# Autodesk Inventor assembly: Euph Mellie Combo Cart
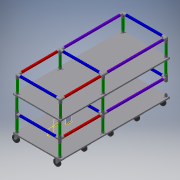
[picture p0: Inventor's stored thumbnail of the model, 180x180]
Saved by Autodesk Inventor 2018.2 (Build 222227000, 227)
## iProperties
Created: 2018-02-07
Part Number: Euph Mellie Combo Cart
Document SubType Name: Assembly
Designer: owner
Author: owner
## Documents named in this file (13)
- Z:\The Pickle\Final Carts\Euph Cart\Euph Mellie Combo Cart.iam
- Z:\The Pickle\Final Carts\Euph Cart\Plywood Base.ipt
- Z:\The Pickle\Inventor Pipe Parts\Formufit Fittings\4-way Tee 1 Inch.ipt
- Z:\The Pickle\Inventor Pipe Parts\Formufit Fittings\Tee 1 Inch.ipt
- Z:\The Pickle\Inventor Pipe Parts\Formufit Fittings\Wood Mount 1 Inch.ipt
- Z:\The Pickle\Final Carts\Euph Cart\Pipe 1.ipt
- Z:\The Pickle\Final Carts\Euph Cart\Pipe 2.ipt
- Z:\The Pickle\Final Carts\Euph Cart\Pipe 3.ipt
- Z:\The Pickle\Final Carts\Euph Cart\Pipe 4.ipt
- Z:\The Pickle\Inventor Pipe Parts\Formufit Fittings\5-way 1 Inch.ipt
- Z:\The Pickle\Inventor Pipe Parts\Formufit Fittings\3-way 90 1 Inch.ipt
- Z:\The Pickle\Final Carts\Eye Bolt and Nut.iam
- Z:\The Pickle\Final Carts\WHEELS.ipt
## Components (76 placed, 12 different names)
1. Plywood Base:1 — Mate:2, Tangent:1, Tangent:2, Tangent:3, Flush:1, Flush:2, Mate:6, Tangent:7, Tangent:8, Tangent:9, Tangent:10, Tangent:11, Mate:14, Flush:36, Flush:37, Flush:38
2. Plywood Base:2 — Mate:3, Mate:4, Tangent:4, Tangent:5, Tangent:6, Flush:1, Flush:2
3. Pipe 1:1 — Insert:47
4. Pipe 1:2 — Insert:48
5. Pipe 1:3 — Insert:41, Insert:42
6. Pipe 1:4 — Insert:9, Insert:10
7. Pipe 1:5 — Insert:11, Insert:12
8. Pipe 1:6 — Insert:3, Insert:4
9. Pipe 2:1 — Insert:45, Insert:46
10. Pipe 2:2 — Insert:37, Insert:38
11. Pipe 2:3 — Insert:5, Insert:6
12. Pipe 3:1 — Insert:13, Insert:30
13. Pipe 3:2 — Insert:14, Insert:33
14. Pipe 3:3 — Insert:1, Insert:2
15. Pipe 3:4 — Insert:15, Insert:34
16. Pipe 3:5 — Insert:17, Insert:31
17. Pipe 3:6 — Insert:18, Insert:26
18. Pipe 3:7 — Insert:16, Insert:32
19. Pipe 3:8 — Insert:19, Insert:29
20. Pipe 3:9 — Insert:21, Insert:27
21. Pipe 3:10 — Insert:20, Insert:25
22. Pipe 3:11 — Insert:22, Insert:28
23. Pipe 3:12 — Insert:23, Insert:24
24. Pipe 4:1 — Insert:39, Insert:40
25. Pipe 4:2 — Insert:7, Insert:8
26. Pipe 4:3 — Insert:43, Insert:44
27. Wood Mount 1 Inch:1 — Insert:54
28. Wood Mount 1 Inch:2 — Insert:34, Tangent:10, Tangent:11
29. Wood Mount 1 Inch:3 — Mate:4, Tangent:4, Tangent:5, Tangent:6, Insert:35
30. Wood Mount 1 Inch:4 — Insert:33
31. Wood Mount 1 Inch:5 — Insert:56
32. Wood Mount 1 Inch:6 — Insert:58
33. Wood Mount 1 Inch:7 — Insert:24, Mate:3
34. Wood Mount 1 Inch:8 — Insert:25
35. Wood Mount 1 Inch:9 — Insert:26
36. Wood Mount 1 Inch:10 — Insert:29
37. Wood Mount 1 Inch:11 — Insert:27
38. Wood Mount 1 Inch:12 — Insert:28, Mate:6, Tangent:7, Tangent:8, Tangent:9
39. Wood Mount 1 Inch:13 — Insert:30
40. Wood Mount 1 Inch:14 — Mate:2, Tangent:1, Tangent:2, Tangent:3, Insert:1
41. Wood Mount 1 Inch:15 — Insert:32
42. Wood Mount 1 Inch:16 — Insert:31
43. Wood Mount 1 Inch:17 — Insert:55
44. Wood Mount 1 Inch:18 — Insert:57
45. 3-way 90 1 Inch:1 — Insert:40, Insert:41, Insert:50
46. 3-way 90 1 Inch:2 — Insert:36, Insert:37
47. 3-way 90 1 Inch:3 — Insert:46, Insert:47, Insert:53
48. 3-way 90 1 Inch:4 — Insert:42, Insert:43, Insert:51
49. 4-way Tee 1 Inch:1 — Insert:38, Insert:39, Insert:49
50. 4-way Tee 1 Inch:2 — Insert:44, Insert:45, Insert:48, Insert:52
51. 4-way Tee 1 Inch:3 — Insert:4, Insert:5, Insert:13, Insert:20
52. 4-way Tee 1 Inch:4 — Insert:8, Insert:9, Insert:15, Insert:21
53. 5-way 1 Inch:2 — Insert:6, Insert:7, Insert:11, Insert:14, Insert:18
54. Tee 1 Inch:1 — Insert:10, Insert:16, Insert:22
55. Tee 1 Inch:2 — Insert:2, Insert:3, Insert:23
56. Tee 1 Inch:3 — Insert:12, Insert:17, Insert:19
57. Pipe 3:13 — Insert:53, Insert:54
58. Pipe 3:14 — Insert:50, Insert:58
59. Pipe 3:15 — Insert:52, Insert:55
60. Pipe 3:16 — Insert:35, Insert:36
61. Pipe 3:17 — Insert:51, Insert:57
62. Pipe 3:18 — Insert:49, Insert:56
63. WHEELS:1 — Flush:14, Flush:15, Flush:17, Flush:38
64. WHEELS:2 — Flush:16, Flush:17, Flush:19, Flush:21
65. WHEELS:3 — Flush:21, Flush:23, Flush:24, Flush:27
66. WHEELS:4 — Flush:26, Flush:27, Flush:29, Flush:32
67. WHEELS:5 — Flush:31, Flush:32, Flush:34
68. WHEELS:6 — Flush:31, Flush:33, Flush:34, Flush:35, Mate:10
69. WHEELS:7 — Flush:26, Flush:28, Flush:29, Flush:30, Flush:33, Flush:35, Mate:10, Mate:11
70. WHEELS:8 — Flush:22, Flush:23, Flush:24, Flush:25, Flush:28, Flush:30, Mate:11, Mate:12
71. WHEELS:9 — Flush:16, Flush:18, Flush:19, Flush:20, Flush:22, Flush:25, Mate:12, Mate:13
72. WHEELS:10 — Flush:14, Flush:15, Flush:18, Flush:20, Mate:13, Mate:14, Flush:36, Flush:37
73. Eye Bolt and Nut:1 [sub-assembly]
74. Eye Bolt and Nut:2 [sub-assembly]
75. Eye Bolt and Nut:3 [sub-assembly]
76. Eye Bolt and Nut:4 [sub-assembly]
## Relationships (105: Insert 58, Flush 27, Tangent 11, Mate 9)
- Mate:2: Plywood Base:1 ↔ Wood Mount 1 Inch:14
- Tangent:1: Plywood Base:1 ↔ Wood Mount 1 Inch:14
- Tangent:2: Plywood Base:1 ↔ Wood Mount 1 Inch:14
- Tangent:3: Plywood Base:1 ↔ Wood Mount 1 Inch:14
- Insert:1: Pipe 3:3 ↔ Wood Mount 1 Inch:14
- Insert:2: Pipe 3:3 ↔ Tee 1 Inch:2
- Insert:3: Pipe 1:6 ↔ Tee 1 Inch:2
- Insert:4: Pipe 1:6 ↔ 4-way Tee 1 Inch:3
- Insert:5: Pipe 2:3 ↔ 4-way Tee 1 Inch:3
- Insert:6: Pipe 2:3 ↔ 5-way 1 Inch:2
- Insert:7: Pipe 4:2 ↔ 5-way 1 Inch:2
- Insert:8: Pipe 4:2 ↔ 4-way Tee 1 Inch:4
- Insert:9: Pipe 1:4 ↔ 4-way Tee 1 Inch:4
- Insert:10: Pipe 1:4 ↔ Tee 1 Inch:1
- Insert:11: Pipe 1:5 ↔ 5-way 1 Inch:2
- Insert:12: Pipe 1:5 ↔ Tee 1 Inch:3
- Insert:13: Pipe 3:1 ↔ 4-way Tee 1 Inch:3
- Insert:14: Pipe 3:2 ↔ 5-way 1 Inch:2
- Insert:15: Pipe 3:4 ↔ 4-way Tee 1 Inch:4
- Insert:16: Pipe 3:7 ↔ Tee 1 Inch:1
- Insert:17: Pipe 3:5 ↔ Tee 1 Inch:3
- Insert:18: Pipe 3:6 ↔ 5-way 1 Inch:2
- Insert:19: Pipe 3:8 ↔ Tee 1 Inch:3
- Insert:20: Pipe 3:10 ↔ 4-way Tee 1 Inch:3
- Insert:21: Pipe 3:9 ↔ 4-way Tee 1 Inch:4
- Insert:22: Pipe 3:11 ↔ Tee 1 Inch:1
- Insert:23: Pipe 3:12 ↔ Tee 1 Inch:2
- Insert:24: Pipe 3:12 ↔ Wood Mount 1 Inch:7
- Insert:25: Pipe 3:10 ↔ Wood Mount 1 Inch:8
- Insert:26: Pipe 3:6 ↔ Wood Mount 1 Inch:9
- Insert:27: Pipe 3:9 ↔ Wood Mount 1 Inch:11
- Insert:28: Pipe 3:11 ↔ Wood Mount 1 Inch:12
- Insert:29: Pipe 3:8 ↔ Wood Mount 1 Inch:10
- Mate:3: Plywood Base:2 ↔ Wood Mount 1 Inch:7
- Insert:30: Pipe 3:1 ↔ Wood Mount 1 Inch:13
- Insert:31: Pipe 3:5 ↔ Wood Mount 1 Inch:16
- Insert:32: Pipe 3:7 ↔ Wood Mount 1 Inch:15
- Insert:33: Pipe 3:2 ↔ Wood Mount 1 Inch:4
- Insert:34: Pipe 3:4 ↔ Wood Mount 1 Inch:2
- Mate:4: Plywood Base:2 ↔ Wood Mount 1 Inch:3
- Tangent:4: Plywood Base:2 ↔ Wood Mount 1 Inch:3
- Tangent:5: Plywood Base:2 ↔ Wood Mount 1 Inch:3
- Tangent:6: Plywood Base:2 ↔ Wood Mount 1 Inch:3
- Insert:35: Wood Mount 1 Inch:3 ↔ Pipe 3:16
- Insert:36: 3-way 90 1 Inch:2 ↔ Pipe 3:16
- Insert:37: Pipe 2:2 ↔ 3-way 90 1 Inch:2
- Insert:38: Pipe 2:2 ↔ 4-way Tee 1 Inch:1
- Insert:39: Pipe 4:1 ↔ 4-way Tee 1 Inch:1
- Insert:40: Pipe 4:1 ↔ 3-way 90 1 Inch:1
- Insert:41: Pipe 1:3 ↔ 3-way 90 1 Inch:1
- Insert:42: Pipe 1:3 ↔ 3-way 90 1 Inch:4
- Insert:43: Pipe 4:3 ↔ 3-way 90 1 Inch:4
- Insert:44: Pipe 4:3 ↔ 4-way Tee 1 Inch:2
- Insert:45: Pipe 2:1 ↔ 4-way Tee 1 Inch:2
- Insert:46: Pipe 2:1 ↔ 3-way 90 1 Inch:3
- Insert:47: Pipe 1:1 ↔ 3-way 90 1 Inch:3
- Insert:48: Pipe 1:2 ↔ 4-way Tee 1 Inch:2
- Insert:49: 4-way Tee 1 Inch:1 ↔ Pipe 3:18
- Insert:50: 3-way 90 1 Inch:1 ↔ Pipe 3:14
- Insert:51: 3-way 90 1 Inch:4 ↔ Pipe 3:17
- Insert:52: 4-way Tee 1 Inch:2 ↔ Pipe 3:15
- Insert:53: 3-way 90 1 Inch:3 ↔ Pipe 3:13
- Insert:54: Wood Mount 1 Inch:1 ↔ Pipe 3:13
- Insert:55: Wood Mount 1 Inch:17 ↔ Pipe 3:15
- Insert:56: Wood Mount 1 Inch:5 ↔ Pipe 3:18
- Insert:57: Wood Mount 1 Inch:18 ↔ Pipe 3:17
- Insert:58: Wood Mount 1 Inch:6 ↔ Pipe 3:14
- Flush:1: Plywood Base:1 ↔ Plywood Base:2
- Flush:2: Plywood Base:1 ↔ Plywood Base:2
- Mate:6: Plywood Base:1 ↔ Wood Mount 1 Inch:12
- Tangent:7: Plywood Base:1 ↔ Wood Mount 1 Inch:12
- Tangent:8: Plywood Base:1 ↔ Wood Mount 1 Inch:12
- Tangent:9: Plywood Base:1 ↔ Wood Mount 1 Inch:12
- Tangent:10: Plywood Base:1 ↔ Wood Mount 1 Inch:2
- Tangent:11: Plywood Base:1 ↔ Wood Mount 1 Inch:2
- Flush:14: WHEELS:1 ↔ WHEELS:10
- Flush:15: WHEELS:1 ↔ WHEELS:10
- Flush:16: WHEELS:2 ↔ WHEELS:9
- Flush:17: WHEELS:1 ↔ WHEELS:2
- Flush:18: WHEELS:9 ↔ WHEELS:10
- Flush:19: WHEELS:2 ↔ WHEELS:9
- Flush:20: WHEELS:9 ↔ WHEELS:10
- Flush:21: WHEELS:2 ↔ WHEELS:3
- Flush:22: WHEELS:8 ↔ WHEELS:9
- Flush:23: WHEELS:3 ↔ WHEELS:8
- Flush:24: WHEELS:3 ↔ WHEELS:8
- Flush:25: WHEELS:8 ↔ WHEELS:9
- Flush:26: WHEELS:4 ↔ WHEELS:7
- Flush:27: WHEELS:3 ↔ WHEELS:4
- Flush:28: WHEELS:7 ↔ WHEELS:8
- Flush:29: WHEELS:4 ↔ WHEELS:7
- Flush:30: WHEELS:7 ↔ WHEELS:8
- Flush:31: WHEELS:5 ↔ WHEELS:6
- Flush:32: WHEELS:4 ↔ WHEELS:5
- Flush:33: WHEELS:6 ↔ WHEELS:7
- Flush:34: WHEELS:5 ↔ WHEELS:6
- Flush:35: WHEELS:6 ↔ WHEELS:7
- Mate:10 (332.7273 mm): WHEELS:6 ↔ WHEELS:7
- Mate:11 (332.7273 mm): WHEELS:7 ↔ WHEELS:8
- Mate:12 (332.7273 mm): WHEELS:8 ↔ WHEELS:9
- Mate:13 (332.7273 mm): WHEELS:9 ↔ WHEELS:10
- Mate:14: Plywood Base:1 ↔ WHEELS:10
- Flush:36: Plywood Base:1 ↔ WHEELS:10
- Flush:37: Plywood Base:1 ↔ WHEELS:10
- Flush:38: Plywood Base:1 ↔ WHEELS:1
